# Autodesk Inventor assembly: Tablero
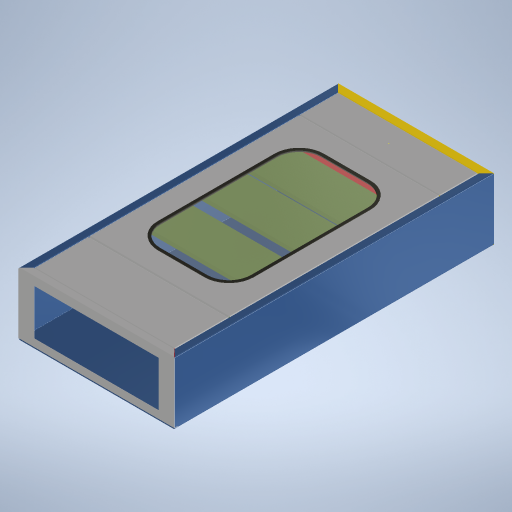
[picture p0: Inventor's stored thumbnail of the model, 512x512]
Saved by Autodesk Inventor 2023 (Build 270158000, 158)
## iProperties
Created: 2022-11-09
Part Number: Tablero
Document SubType Name: Assembly
Designer: David
Author: David
## Documents named in this file (12)
- C:\Users\andre\Downloads\Computacion Grafica\main\Tableros\Tablero.iam
- C:\Users\andre\Downloads\Computacion Grafica\main\Tableros\Tapa_Superior.ipt
- C:\Users\andre\Downloads\Computacion Grafica\main\Tableros\tapa_trasera.ipt
- C:\Users\andre\Downloads\Computacion Grafica\main\Tableros\Divisor.ipt
- C:\Users\andre\Downloads\Computacion Grafica\main\Tableros\Acoplador_de_Cuentas.ipt
- C:\Users\andre\Downloads\Computacion Grafica\main\Tableros\Tapa inferior.ipt
- C:\Users\andre\Downloads\Computacion Grafica\main\Tableros\TapaDown.ipt
- C:\Users\andre\Downloads\Computacion Grafica\main\Tableros\TapaUp.ipt
- C:\Users\andre\Downloads\Computacion Grafica\main\Tableros\TapaCentral.ipt
- C:\Users\andre\Downloads\Computacion Grafica\main\Tableros\Caucho.ipt
- C:\Users\andre\Downloads\Computacion Grafica\main\Tableros\PLatico.ipt
- C:\Users\andre\Downloads\Computacion Grafica\main\Tableros\datos.xlsx
## Components (17 placed, 10 different names)
1. Tapa_Superior:1 — Flush:1, Mate:1, Flush:2, Mate:21, Mate:23
2. tapa_trasera:1 — Flush:1, Mate:1, Flush:2, Mate:2, Mate:3, Mate:5, Flush:3, Mate:7, Flush:4, Mate:9, Flush:5, Mate:11, Mate:12, Mate:13, Mate:14, Mate:15, Mate:16, Mate:17, Mate:18, Mate:19, Mate:20, Mate:22, Flush:12, Mate:24, Flush:13, Mate:25, Flush:14, Flush:15, Mate:26, Flush:16, Mate:28
3. Divisor:1 — Mate:2, Mate:3, Mate:10, Mate:21
4. Divisor:2 — Mate:5, Flush:3, Mate:22
5. Acoplador_de_Cuentas:1 — Mate:9, Flush:5, Mate:10, Flush:6
6. Acoplador_de_Cuentas:2 — Mate:7, Flush:4, Flush:6, Flush:7
7. Acoplador_de_Cuentas:3 — Mate:11, Mate:12, Flush:7, Flush:8
8. Acoplador_de_Cuentas:4 — Mate:14, Mate:18, Flush:8, Flush:9
9. Acoplador_de_Cuentas:5 — Mate:13, Mate:17, Flush:9, Flush:10
10. Acoplador_de_Cuentas:6 — Mate:15, Mate:19, Flush:10, Flush:11
11. Acoplador_de_Cuentas:7 — Mate:16, Mate:20, Flush:11
12. TapaDown:1 — Flush:15, Mate:26, Mate:27
13. TapaUp:1 — Flush:12, Mate:23, Mate:24, Mate:29
14. Tapa inferior:1 — Flush:13, Mate:25, Flush:14, Mate:27
15. TapaCentral:1 — Flush:16, Mate:28, Mate:29, Mate:30, Mate:31, Mate:32
16. Caucho:1 — Mate:30, Mate:31, Mate:32, Mate:33, Mate:34, Mate:35
17. PLatico:1 — Mate:33, Mate:34, Mate:35
## Relationships (48: Mate 32, Flush 16)
- Flush:1: Tapa_Superior:1 ↔ tapa_trasera:1
- Mate:1: Tapa_Superior:1 ↔ tapa_trasera:1
- Flush:2: Tapa_Superior:1 ↔ tapa_trasera:1
- Mate:2: tapa_trasera:1 ↔ Divisor:1
- Mate:3: tapa_trasera:1 ↔ Divisor:1
- Mate:5: tapa_trasera:1 ↔ Divisor:2
- Flush:3 (400 mm): tapa_trasera:1 ↔ Divisor:2
- Mate:7: tapa_trasera:1 ↔ Acoplador_de_Cuentas:2
- Flush:4 (220 mm): tapa_trasera:1 ↔ Acoplador_de_Cuentas:2
- Mate:9: tapa_trasera:1 ↔ Acoplador_de_Cuentas:1
- Flush:5 (220 mm): tapa_trasera:1 ↔ Acoplador_de_Cuentas:1
- Mate:10 (150 mm): Divisor:1 ↔ Acoplador_de_Cuentas:1
- Flush:6 (300 mm): Acoplador_de_Cuentas:1 ↔ Acoplador_de_Cuentas:2
- Mate:11: tapa_trasera:1 ↔ Acoplador_de_Cuentas:3
- Mate:12 (-220 mm): tapa_trasera:1 ↔ Acoplador_de_Cuentas:3
- Mate:13: tapa_trasera:1 ↔ Acoplador_de_Cuentas:5
- Mate:14: tapa_trasera:1 ↔ Acoplador_de_Cuentas:4
- Mate:15: tapa_trasera:1 ↔ Acoplador_de_Cuentas:6
- Mate:16: tapa_trasera:1 ↔ Acoplador_de_Cuentas:7
- Mate:17 (-220 mm): tapa_trasera:1 ↔ Acoplador_de_Cuentas:5
- Mate:18 (-220 mm): tapa_trasera:1 ↔ Acoplador_de_Cuentas:4
- Mate:19 (-220 mm): tapa_trasera:1 ↔ Acoplador_de_Cuentas:6
- Mate:20 (-220 mm): tapa_trasera:1 ↔ Acoplador_de_Cuentas:7
- Flush:7 (350 mm): Acoplador_de_Cuentas:2 ↔ Acoplador_de_Cuentas:3
- Flush:8 (350 mm): Acoplador_de_Cuentas:3 ↔ Acoplador_de_Cuentas:4
- Flush:9 (175 mm): Acoplador_de_Cuentas:4 ↔ Acoplador_de_Cuentas:5
- Flush:10: Acoplador_de_Cuentas:5 ↔ Acoplador_de_Cuentas:6
- Flush:11: Acoplador_de_Cuentas:6 ↔ Acoplador_de_Cuentas:7
- Mate:21 (300 mm): Tapa_Superior:1 ↔ Divisor:1
- Mate:22: tapa_trasera:1 ↔ Divisor:2
- Flush:12: tapa_trasera:1 ↔ TapaUp:1
- Mate:23: Tapa_Superior:1 ↔ TapaUp:1
- Mate:24: tapa_trasera:1 ↔ TapaUp:1
- Flush:13: tapa_trasera:1 ↔ Tapa inferior:1
- Mate:25: tapa_trasera:1 ↔ Tapa inferior:1
- Flush:14: tapa_trasera:1 ↔ Tapa inferior:1
- Flush:15: tapa_trasera:1 ↔ TapaDown:1
- Mate:26: tapa_trasera:1 ↔ TapaDown:1
- Mate:27: TapaDown:1 ↔ Tapa inferior:1
- Flush:16: tapa_trasera:1 ↔ TapaCentral:1
- Mate:28: tapa_trasera:1 ↔ TapaCentral:1
- Mate:29: TapaUp:1 ↔ TapaCentral:1
- Mate:30: TapaCentral:1 ↔ Caucho:1
- Mate:31: TapaCentral:1 ↔ Caucho:1
- Mate:32: TapaCentral:1 ↔ Caucho:1
- Mate:33: Caucho:1 ↔ PLatico:1
- Mate:34: Caucho:1 ↔ PLatico:1
- Mate:35: Caucho:1 ↔ PLatico:1
## Named parameters: SpaceDown = 400 mm, SpaceFront = 220 mm, Bandejas = 4, Alto = 2050 mm, Ancho = 1000 mm, Space1 = 250 mm, Space2 = 350 mm, Space3 = 350 mm, Space4 = 350 mm, Space5 = 0 mm, Space6 = 0 mm, Space7 = 0 mm, iTrigger0 = 3
